# Autodesk Inventor assembly: new_ㄷ_frame
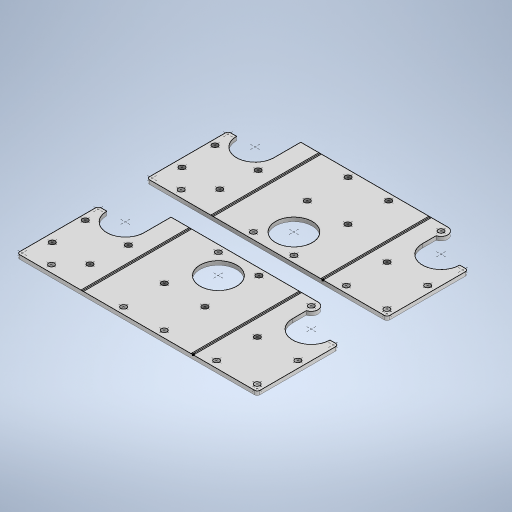
[picture p0: Inventor's stored thumbnail of the model, 512x512]
Saved by Autodesk Inventor 2024.2 (Build 282272000, 272)
## iProperties
Created: 2024-01-14
Part Number: new_ㄷ_frame
Document SubType Name: Assembly
Designer: chanh
Author: chanh
## Documents named in this file (3)
- C:\Users\chanh\내 드라이브\로봇\Humanoid\Roboin Humanoid Project\Inventor\rh_plus_7_axis_robot_arm_hardware\CAM\1.5T\new_ㄷ_frame\new_ㄷ_frame.iam
- C:\Users\chanh\내 드라이브\로봇\Humanoid\Roboin Humanoid Project\Inventor\rh_plus_7_axis_robot_arm_hardware\CAM\1.5T\new_ㄷ_frame\axis_3_top_frame.ipt
- C:\Users\chanh\내 드라이브\로봇\Humanoid\Roboin Humanoid Project\Inventor\rh_plus_7_axis_robot_arm_hardware\CAM\1.5T\new_ㄷ_frame\axis_5_top_frame.ipt
## Components (2 placed, 2 different names)
1. axis_3_top_frame:1 — Mate:3, Flush:2, Flush:3
2. axis_5_top_frame:1 — Mate:1, Flush:1, Mate:2, Mate:3, Flush:2, Flush:3
## Relationships (6: Mate 3, Flush 3)
- Mate:1: axis_5_top_frame:1
- Flush:1: axis_5_top_frame:1
- Mate:2: axis_5_top_frame:1
- Mate:3 (8 mm): axis_3_top_frame:1 ↔ axis_5_top_frame:1
- Flush:2: axis_3_top_frame:1 ↔ axis_5_top_frame:1
- Flush:3: axis_3_top_frame:1 ↔ axis_5_top_frame:1
